# Autodesk Inventor assembly: Gertiebe
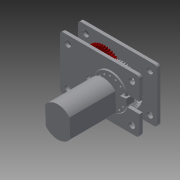
[picture p0: Inventor's stored thumbnail of the model, 180x180]
Saved by Autodesk Inventor 2014 (Build 180170000, 170)
## iProperties
Created: 2013-05-31
Part Number: Gertiebe
Document SubType Name: Assembly
Designer: hanse
Author: hanse
## Documents named in this file (9)
- C:\Users\hanse\Desktop\Beep\Hardware\GetriebeB\GertiebeBCNCld.iam
- C:\Users\hanse\Desktop\Beep\Hardware\GetriebeB\Gertiebe\Konstruktions-Assistent\Stirnräder3.iam
- C:\Users\hanse\Desktop\Beep\Hardware\GetriebeB\DoppelZahnrad.iam
- C:\Users\hanse\Desktop\Beep\Hardware\EE-SX1131.ipt
- C:\Users\hanse\Desktop\Beep\Hardware\GetriebeB\EncoderWheel2.ipt
- C:\Users\hanse\Desktop\Beep\Hardware\GetriebeB\DopelZahnrad\Konstruktions-Assistent\Stirnzahnrad21.ipt
- C:\Users\hanse\Desktop\Beep\Hardware\GetriebeB\frontcncld.ipt
- C:\Users\hanse\Desktop\Beep\Hardware\GetriebeB\backcncld.ipt
- C:\Users\hanse\Desktop\Beep\Hardware\Model1\motor.ipt
## Components (9 placed, 8 different names)
1. Stirnräder:3 [sub-assembly] — Passend:2, Passend:8, Passend:13, Passend:21
2. DoppelZahnrad:2 [sub-assembly] — Passend:2, Passend:8, Passend:19, Passend:20
3. DoppelZahnrad:3 [sub-assembly] — Passend:15, Passend:16, Passend:22
4. EE-SX1131:1 — Passend:14, Tangential:1
5. EncoderWheel2:1 — Passend:13, Passend:14, Passend:21, Passend:23, Tangential:1
6. Stirnzahnrad2:1 — Passend:15, Passend:16, Passend:17, Passend:18
7. frontcncld:1 — Passend:17, Passend:18, Passend:19, Passend:20
8. backcncld:1 — Passend:22
9. motor:1 — Passend:23
## Relationships (14: Mate 13, Tangent 1)
- Passend:2 [Mate]: Stirnräder:3 ↔ DoppelZahnrad:2
- Passend:8 [Mate]: Stirnräder:3 ↔ DoppelZahnrad:2
- Passend:13 [Mate]: Stirnräder:3 ↔ EncoderWheel2:1
- Passend:14 [Mate] (0.05 mm): EE-SX1131:1 ↔ EncoderWheel2:1
- Passend:15 [Mate]: DoppelZahnrad:3 ↔ Stirnzahnrad2:1
- Passend:16 [Mate]: DoppelZahnrad:3 ↔ Stirnzahnrad2:1
- Passend:17 [Mate]: Stirnzahnrad2:1 ↔ frontcncld:1
- Passend:18 [Mate]: Stirnzahnrad2:1 ↔ frontcncld:1
- Passend:19 [Mate]: DoppelZahnrad:2 ↔ frontcncld:1
- Passend:20 [Mate]: DoppelZahnrad:2 ↔ frontcncld:1
- Passend:21 [Mate]: Stirnräder:3 ↔ EncoderWheel2:1
- Passend:22 [Mate]: DoppelZahnrad:3 ↔ backcncld:1
- Passend:23 [Mate]: EncoderWheel2:1 ↔ motor:1
- Tangential:1: EE-SX1131:1 ↔ EncoderWheel2:1
